# Autodesk Inventor assembly: A1200 Keyboard
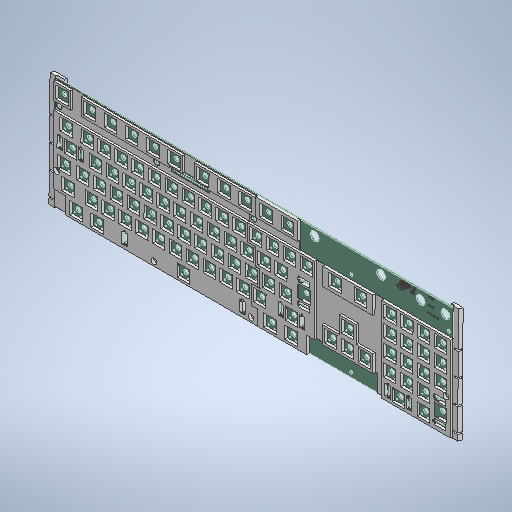
[picture p0: Inventor's stored thumbnail of the model, 512x512]
Saved by Autodesk Inventor 2025 (Build 290162000, 162)
## iProperties
Created: 2024-08-20
Part Number: A1200 Keyboard
Document SubType Name: Assembly
Designer: adam
Author: adam
## Documents named in this file (6)
- C:\Users\adam\Projects\A1200KBv2\3dprint\Keyboard plates\A1200 Keyboard.iam
- C:\Users\adam\Projects\A1200KBv2\3dprint\Keyboard plates\A1200KBv2r5\A1200KBv2r5.ipt
- C:\Users\adam\Projects\A1200KBv2\3dprint\A1200net\Mounting\A1200net Left mount.ipt
- C:\Users\adam\Projects\A1200KBv2\3dprint\A1200net\Mounting\A1200net Right mount.ipt
- C:\Users\adam\Projects\A1200KBv2\3dprint\Keyboard plates\Left Plate.ipt
- C:\Users\adam\Projects\A1200KBv2\3dprint\Keyboard plates\Right Plate.ipt
## Components (5 placed, 5 different names)
1. A1200KBv2r5:1 — Mate:1, Mate:2, Mate:3, Mate:4, Flush:1, Flush:2
2. A1200net Left mount:1 — Mate:1, Mate:2
3. A1200net Right mount:1 — Mate:3, Mate:4
4. Left Plate:1 — Flush:1
5. Right Plate:1 — Flush:2
## Relationships (6: Mate 4, Flush 2)
- Mate:1: A1200KBv2r5:1 ↔ A1200net Left mount:1
- Mate:2: A1200KBv2r5:1 ↔ A1200net Left mount:1
- Mate:3: A1200KBv2r5:1 ↔ A1200net Right mount:1
- Mate:4: A1200KBv2r5:1 ↔ A1200net Right mount:1
- Flush:1: A1200KBv2r5:1 ↔ Left Plate:1
- Flush:2: A1200KBv2r5:1 ↔ Right Plate:1
